# Autodesk Inventor assembly: Body_Modified
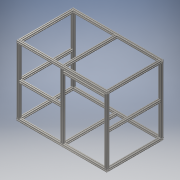
[picture p0: Inventor's stored thumbnail of the model, 180x180]
Saved by Autodesk Inventor 2019 (Build 230136000, 136)
## iProperties
Created: 2019-04-11
Part Number: Body_Modified
Material: 일반
Document SubType Name: Assembly
Designer: hinmo
Mass: 3617.53 g
Surface Area: 107255 cm^2
Volume: 401340 cm^3
Density: 0.00901363 g/cm^3
Author: hinmo
## Documents named in this file (5)
- C:\Users\hinmo\Documents\Inventor\Projects\2019_CapstoneDesign\Body_Modified.iam
- C:\Users\hinmo\Documents\Inventor\Projects\2019_CapstoneDesign\Propile_50.ipt
- C:\Users\hinmo\Documents\Inventor\Projects\2019_CapstoneDesign\Propile_70.ipt
- C:\Users\hinmo\Documents\Inventor\Projects\2019_CapstoneDesign\Propile_37.ipt
- C:\Users\hinmo\Documents\Inventor\Projects\2019_CapstoneDesign\Propile_32.ipt
## Components (19 placed, 4 different names)
1. Propile_50:1 — 메이트:5, 플러쉬:2, 메이트:7, 플러쉬:3, 플러쉬:10, 플러쉬:11, 플러쉬:29
2. Propile_50:2 — 메이트:12, 플러쉬:14, 플러쉬:15, 플러쉬:18, 플러쉬:19, 메이트:25, 플러쉬:26, 메이트:32
3. Propile_50:3 — 메이트:3, 플러쉬:1, 메이트:18, 플러쉬:30
4. Propile_50:4 — 메이트:13, 메이트:14, 메이트:15, 플러쉬:12, 플러쉬:13, 플러쉬:16, 플러쉬:17, 메이트:23, 플러쉬:27
5. Propile_70:1 — 메이트:7, 플러쉬:3, 메이트:9, 메이트:11, 플러쉬:7, 플러쉬:8, 플러쉬:9, 메이트:21, 메이트:31
6. Propile_70:2 — 메이트:14, 플러쉬:13, 플러쉬:14, 플러쉬:17, 플러쉬:18, 메이트:16, 플러쉬:20, 플러쉬:21, 메이트:24, 메이트:30
7. Propile_70:3 — 메이트:12, 메이트:13, 메이트:15, 플러쉬:12, 플러쉬:15, 플러쉬:16, 플러쉬:19, 메이트:22, 플러쉬:28, 메이트:33
8. Propile_70:4 — 메이트:3, 플러쉬:1, 메이트:5, 플러쉬:2, 메이트:8, 플러쉬:4, 플러쉬:5, 메이트:10, 플러쉬:6, 메이트:17, 플러쉬:22
9. Propile_37:1 — 메이트:8, 플러쉬:4, 플러쉬:5, 플러쉬:20, 플러쉬:21, 메이트:29
10. Propile_37:2 — 메이트:9, 플러쉬:8, 플러쉬:9, 메이트:27
11. Propile_37:3 — 메이트:10, 플러쉬:6, 플러쉬:11, 메이트:26, 플러쉬:25, 메이트:28, 메이트:30
12. Propile_37:4 — 메이트:11, 플러쉬:7, 플러쉬:10, 메이트:16
13. Propile_50:5 — 메이트:17, 플러쉬:22, 메이트:18, 메이트:19, 메이트:20, 플러쉬:23, 플러쉬:24
14. Propile_32:1 — 메이트:19, 플러쉬:24, 메이트:21, 플러쉬:29
15. Propile_32:2 — 메이트:20, 플러쉬:23, 플러쉬:30
16. Propile_37:5 — 메이트:25, 플러쉬:26, 메이트:28
17. Propile_37:6 — 메이트:22, 메이트:27, 플러쉬:28
18. Propile_37:7 — 메이트:23, 플러쉬:27, 메이트:29
19. Propile_37:8 — 메이트:24, 메이트:26, 플러쉬:25
## Relationships (59: Flush 30, Mate 29)
- 메이트:3 [Mate]: Propile_50:3 ↔ Propile_70:4
- 플러쉬:1 [Flush]: Propile_50:3 ↔ Propile_70:4
- 메이트:5 [Mate]: Propile_50:1 ↔ Propile_70:4
- 플러쉬:2 [Flush]: Propile_50:1 ↔ Propile_70:4
- 메이트:7 [Mate]: Propile_50:1 ↔ Propile_70:1
- 플러쉬:3 [Flush]: Propile_50:1 ↔ Propile_70:1
- 메이트:8 [Mate]: Propile_70:4 ↔ Propile_37:1
- 플러쉬:4 [Flush]: Propile_70:4 ↔ Propile_37:1
- 플러쉬:5 [Flush]: Propile_70:4 ↔ Propile_37:1
- 메이트:9 [Mate]: Propile_70:1 ↔ Propile_37:2
- 메이트:10 [Mate]: Propile_70:4 ↔ Propile_37:3
- 메이트:11 [Mate]: Propile_70:1 ↔ Propile_37:4
- 플러쉬:6 [Flush]: Propile_70:4 ↔ Propile_37:3
- 플러쉬:7 [Flush]: Propile_70:1 ↔ Propile_37:4
- 플러쉬:8 [Flush]: Propile_70:1 ↔ Propile_37:2
- 플러쉬:9 [Flush]: Propile_70:1 ↔ Propile_37:2
- 플러쉬:10 [Flush]: Propile_50:1 ↔ Propile_37:4
- 플러쉬:11 [Flush]: Propile_50:1 ↔ Propile_37:3
- 메이트:12 [Mate]: Propile_50:2 ↔ Propile_70:3
- 메이트:13 [Mate]: Propile_50:4 ↔ Propile_70:3
- 메이트:14 [Mate]: Propile_50:4 ↔ Propile_70:2
- 메이트:15 [Mate]: Propile_50:4 ↔ Propile_70:3
- 플러쉬:12 [Flush]: Propile_50:4 ↔ Propile_70:3
- 플러쉬:13 [Flush]: Propile_50:4 ↔ Propile_70:2
- 플러쉬:14 [Flush]: Propile_50:2 ↔ Propile_70:2
- 플러쉬:15 [Flush]: Propile_50:2 ↔ Propile_70:3
- 플러쉬:16 [Flush]: Propile_50:4 ↔ Propile_70:3
- 플러쉬:17 [Flush]: Propile_50:4 ↔ Propile_70:2
- 플러쉬:18 [Flush]: Propile_50:2 ↔ Propile_70:2
- 플러쉬:19 [Flush]: Propile_50:2 ↔ Propile_70:3
- 메이트:16 [Mate]: Propile_70:2 ↔ Propile_37:4
- 플러쉬:20 [Flush]: Propile_70:2 ↔ Propile_37:1
- 플러쉬:21 [Flush]: Propile_70:2 ↔ Propile_37:1
- 메이트:17 [Mate]: Propile_70:4 ↔ Propile_50:5
- 플러쉬:22 [Flush]: Propile_70:4 ↔ Propile_50:5
- 메이트:18 [Mate] (320 mm): Propile_50:3 ↔ Propile_50:5
- 메이트:19 [Mate]: Propile_50:5 ↔ Propile_32:1
- 메이트:20 [Mate]: Propile_50:5 ↔ Propile_32:2
- 플러쉬:23 [Flush]: Propile_50:5 ↔ Propile_32:2
- 플러쉬:24 [Flush]: Propile_50:5 ↔ Propile_32:1
- 메이트:21 [Mate] (240 mm): Propile_70:1 ↔ Propile_32:1
- 메이트:22 [Mate]: Propile_70:3 ↔ Propile_37:6
- 메이트:23 [Mate]: Propile_50:4 ↔ Propile_37:7
- 메이트:24 [Mate]: Propile_70:2 ↔ Propile_37:8
- 메이트:25 [Mate]: Propile_50:2 ↔ Propile_37:5
- 메이트:26 [Mate] (320 mm): Propile_37:3 ↔ Propile_37:8
- 메이트:27 [Mate] (320 mm): Propile_37:2 ↔ Propile_37:6
- 플러쉬:25 [Flush]: Propile_37:3 ↔ Propile_37:8
- 플러쉬:26 [Flush]: Propile_50:2 ↔ Propile_37:5
- 플러쉬:27 [Flush]: Propile_50:4 ↔ Propile_37:7
- 플러쉬:28 [Flush]: Propile_70:3 ↔ Propile_37:6
- 메이트:28 [Mate] (240 mm): Propile_37:3 ↔ Propile_37:5
- 메이트:29 [Mate] (240 mm): Propile_37:1 ↔ Propile_37:7
- 메이트:30 [Mate]: Propile_70:2 ↔ Propile_37:3
- 플러쉬:29 [Flush]: Propile_50:1 ↔ Propile_32:1
- 플러쉬:30 [Flush]: Propile_50:3 ↔ Propile_32:2
- 메이트:31 [Mate]: Propile_70:1
- 메이트:32 [Mate]: Propile_50:2
- 메이트:33 [Mate]: Propile_70:3
